# Autodesk Inventor assembly: Assembly1
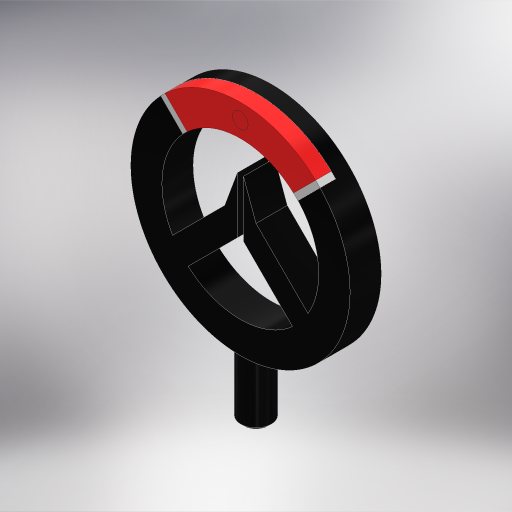
[picture p0: Inventor's stored thumbnail of the model, 512x512]
Saved by Autodesk Inventor 2024 (Build 280153000, 153)
## iProperties
Created: 2023-10-30
Part Number: Assembly1
Document SubType Name: Assembly
Designer: SSAFY
Author: SSAFY
## Documents named in this file (5)
- C:\Users\SSAFY\Desktop\TIL\3D\20231030\Assembly1.iam
- C:\Users\SSAFY\Desktop\TIL\3D\20231030\Black_Part1.ipt
- C:\Users\SSAFY\Desktop\TIL\3D\20231030\Red_part1.ipt
- C:\Users\SSAFY\Desktop\TIL\3D\20231030\White_Part1.ipt
- C:\Users\SSAFY\Desktop\TIL\3D\20231030\Red_Part2.ipt
## Components (5 placed, 4 different names)
1. Black_Part1:2 — Mate:6, Mate:7
2. Red_part1:1 — Mate:1, Mate:2, Flush:1, Mate:3, Flush:2, Mate:4, Flush:3, Mate:5, Mate:6
3. White_Part1:1 — Mate:1, Mate:2, Flush:1
4. White_Part1:2 — Mate:3, Flush:2, Mate:4
5. Red_Part2:1 — Flush:3, Mate:5, Mate:7
## Relationships (10: Mate 7, Flush 3)
- Mate:1: Red_part1:1 ↔ White_Part1:1
- Mate:2: Red_part1:1 ↔ White_Part1:1
- Flush:1: Red_part1:1 ↔ White_Part1:1
- Mate:3: Red_part1:1 ↔ White_Part1:2
- Flush:2: Red_part1:1 ↔ White_Part1:2
- Mate:4: Red_part1:1 ↔ White_Part1:2
- Flush:3: Red_part1:1 ↔ Red_Part2:1
- Mate:5: Red_part1:1 ↔ Red_Part2:1
- Mate:6: Black_Part1:2 ↔ Red_part1:1
- Mate:7: Black_Part1:2 ↔ Red_Part2:1
